# Autodesk Inventor assembly: Baterías
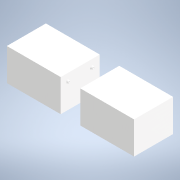
[picture p0: Inventor's stored thumbnail of the model, 180x180]
Saved by Autodesk Inventor 2022.1 (Build 261234000, 234)
## iProperties
Created: 2021-10-01
Part Number: Baterías
Document SubType Name: Assembly
Designer: seb_0
Mass: 33006.4 g
Surface Area: 8204.7 cm^2
Volume: 18507.6 cm^3
Density: 1.7834 g/cm^3
Author: seb_0
## Documents named in this file (2)
- C:\Users\seb_0\Desktop\PDM\ProyectoRobotPallet\Batería\Baterías.iam
- C:\Users\seb_0\Desktop\PDM\ProyectoRobotPallet\Batería\Batería.ipt
## Components (2 placed, 1 different names)
1. Batería:1 — Coincidencia:1, Coincidencia:2, Nivelación:1, Coincidencia:3, Nivelación:2
2. Batería:2 — Nivelación:1, Coincidencia:3, Nivelación:2
## Relationships (5: Mate 3, Flush 2)
- Coincidencia:1 [Mate]: Batería:1
- Coincidencia:2 [Mate]: Batería:1
- Nivelación:1 [Flush]: Batería:1 ↔ Batería:2
- Coincidencia:3 [Mate] (100 mm): Batería:1 ↔ Batería:2
- Nivelación:2 [Flush]: Batería:1 ↔ Batería:2
